# Autodesk Inventor assembly: RUKA ROBOT ASSEMBLY
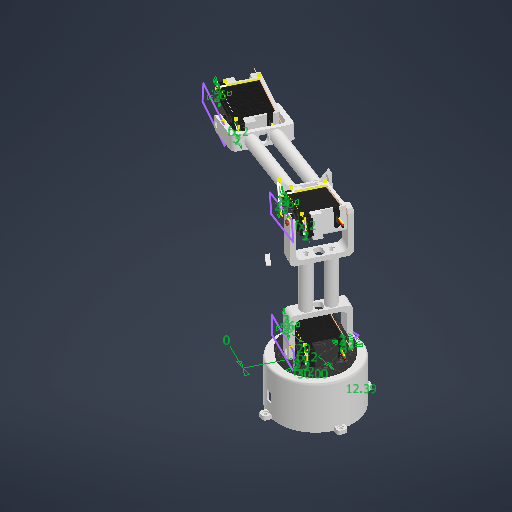
[picture p0: Inventor's stored thumbnail of the model, 512x512]
Saved by Autodesk Inventor 2026 (Build 300175000, 175)
## iProperties
Created: 2025-04-11
Part Number: RUKA ROBOT ASSEMBLY
Document SubType Name: Assembly
Designer: janpa
Author: janpa
## Documents named in this file (11)
- C:\Users\janpa\OneDrive\Plocha\Hackaton\Hackathon25\3d\RUKA ROBOT ASSEMBLY.iam
- C:\Users\janpa\Downloads\MG995-Servo.ipt
- C:\Users\janpa\OneDrive\Plocha\Hackaton\Hackathon25\3d\ruka base.ipt
- C:\Users\janpa\OneDrive\Plocha\Hackaton\Hackathon25\3d\rotacniZaklad.ipt
- C:\Users\janpa\OneDrive\Plocha\Hackaton\Hackathon25\3d\ruka_part spodni.ipt
- C:\Users\janpa\OneDrive\Plocha\Hackaton\Hackathon25\3d\extendo1.ipt
- C:\Users\janpa\OneDrive\Plocha\Hackaton\Hackathon25\3d\servo_horni_kloub.ipt
- C:\Users\janpa\OneDrive\Plocha\Hackaton\Hackathon25\3d\horni_kloub_extenze_drzak.ipt
- C:\Users\janpa\OneDrive\Plocha\Hackaton\Hackathon25\3d\valec_3mm.ipt
- C:\Users\janpa\OneDrive\Plocha\Hackaton\Hackathon25\3d\extendo100.ipt
- C:\Users\janpa\OneDrive\Plocha\Hackaton\Hackathon25\3d\BLOK.ipt
## Components (18 placed, 10 different names)
1. MG995-Servo:1 — Mate:1, Mate:2, Mate:4
2. ruka base:1 — Mate:1, Mate:5
3. rotacniZaklad:1 — Mate:2, Mate:4, Mate:5, Mate:6, Mate:7, Mate:8
4. MG995-Servo:2 — Mate:6, Mate:7, Mate:8, Mate:9, Mate:10
5. ruka_part spodni:1 — Mate:9, Mate:10, Mate:11, Mate:12, Mate:13, Mate:14
6. extendo1:1 — Mate:11, Mate:12, Mate:16, Mate:17
7. extendo1:2 — Mate:13, Mate:14, Mate:15, Mate:18
8. ruka_part spodni:2 — Mate:15, Mate:16, Mate:17, Mate:18, Mate:22, Mate:23
9. MG995-Servo:3 — Mate:19, Mate:20, Mate:21, Mate:23, Mate:24, Mate:31
10. servo_horni_kloub:1 — Mate:19, Mate:20, Mate:21, Mate:22, Mate:25, Mate:42
11. horni_kloub_extenze_drzak:1 — Mate:24, Mate:25, Mate:26, Mate:27, Mate:28, Mate:29, Mate:30, Mate:43
12. extendo100:1 — Mate:28, Mate:29, Mate:33, Mate:35
13. extendo100:2 — Mate:26, Mate:27, Mate:32, Mate:34
14. valec_3mm:1 — Mate:30, Mate:31
15. ruka_part spodni:4 — Mate:32, Mate:33, Mate:34, Mate:35, Mate:36, Mate:40
16. servo_horni_kloub:2 — Mate:36, Mate:37, Mate:38, Mate:39, Mate:41
17. MG995-Servo:4 — Mate:37, Mate:38, Mate:39, Mate:40, Mate:41
18. BLOK:1 — Mate:42, Mate:43
## Relationships (42: Mate 42)
- Mate:1: MG995-Servo:1 ↔ ruka base:1
- Mate:2: MG995-Servo:1 ↔ rotacniZaklad:1
- Mate:4: MG995-Servo:1 ↔ rotacniZaklad:1
- Mate:5: ruka base:1 ↔ rotacniZaklad:1
- Mate:6: rotacniZaklad:1 ↔ MG995-Servo:2
- Mate:7: rotacniZaklad:1 ↔ MG995-Servo:2
- Mate:8: rotacniZaklad:1 ↔ MG995-Servo:2
- Mate:9: MG995-Servo:2 ↔ ruka_part spodni:1
- Mate:10: MG995-Servo:2 ↔ ruka_part spodni:1
- Mate:11: ruka_part spodni:1 ↔ extendo1:1
- Mate:12: ruka_part spodni:1 ↔ extendo1:1
- Mate:13: ruka_part spodni:1 ↔ extendo1:2
- Mate:14: ruka_part spodni:1 ↔ extendo1:2
- Mate:15: extendo1:2 ↔ ruka_part spodni:2
- Mate:16: extendo1:1 ↔ ruka_part spodni:2
- Mate:17: extendo1:1 ↔ ruka_part spodni:2
- Mate:18: extendo1:2 ↔ ruka_part spodni:2
- Mate:19: MG995-Servo:3 ↔ servo_horni_kloub:1
- Mate:20: MG995-Servo:3 ↔ servo_horni_kloub:1
- Mate:21: MG995-Servo:3 ↔ servo_horni_kloub:1
- Mate:22: ruka_part spodni:2 ↔ servo_horni_kloub:1
- Mate:23: ruka_part spodni:2 ↔ MG995-Servo:3
- Mate:24: MG995-Servo:3 ↔ horni_kloub_extenze_drzak:1
- Mate:25: servo_horni_kloub:1 ↔ horni_kloub_extenze_drzak:1
- Mate:26: horni_kloub_extenze_drzak:1 ↔ extendo100:2
- Mate:27: horni_kloub_extenze_drzak:1 ↔ extendo100:2
- Mate:28: horni_kloub_extenze_drzak:1 ↔ extendo100:1
- Mate:29: horni_kloub_extenze_drzak:1 ↔ extendo100:1
- Mate:30: horni_kloub_extenze_drzak:1 ↔ valec_3mm:1
- Mate:31: MG995-Servo:3 ↔ valec_3mm:1
- Mate:32: extendo100:2 ↔ ruka_part spodni:4
- Mate:33: extendo100:1 ↔ ruka_part spodni:4
- Mate:34: extendo100:2 ↔ ruka_part spodni:4
- Mate:35: extendo100:1 ↔ ruka_part spodni:4
- Mate:36: ruka_part spodni:4 ↔ servo_horni_kloub:2
- Mate:37: servo_horni_kloub:2 ↔ MG995-Servo:4
- Mate:38: servo_horni_kloub:2 ↔ MG995-Servo:4
- Mate:39: servo_horni_kloub:2 ↔ MG995-Servo:4
- Mate:40: ruka_part spodni:4 ↔ MG995-Servo:4
- Mate:41: servo_horni_kloub:2 ↔ MG995-Servo:4
- Mate:42: servo_horni_kloub:1 ↔ BLOK:1
- Mate:43: horni_kloub_extenze_drzak:1 ↔ BLOK:1
